# Autodesk Inventor assembly: MaleHeader-02
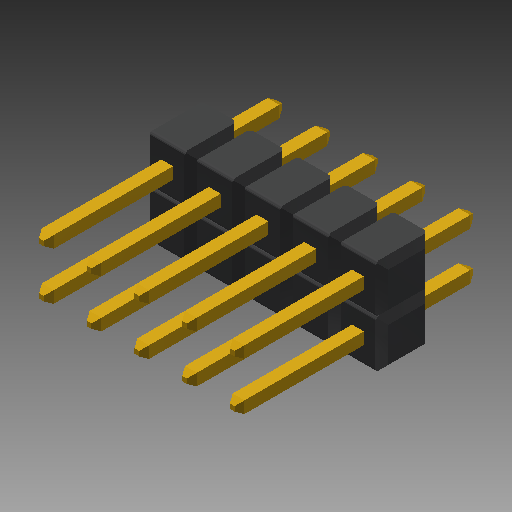
[picture p0: Inventor's stored thumbnail of the model, 512x512]
Saved by Autodesk Inventor 2018 (Build 220112000, 112)
## iProperties
Created: 2017-04-09
Part Number: MaleHeader-02
Document SubType Name: Assembly
Designer: dkt01
Author: dkt01
## Documents named in this file (2)
- C:\Users\dktur\Dropbox\StackLightMonitor\CAD\MaleHeader-02.iam
- C:\Users\dktur\Dropbox\StackLightMonitor\CAD\MaleHeader-02.ipt
## Components (10 placed, 1 different names)
1. MaleHeader-02:1
2. MaleHeader-02:2
3. MaleHeader-02:3
4. MaleHeader-02:4
5. MaleHeader-02:5
6. MaleHeader-02:6
7. MaleHeader-02:7
8. MaleHeader-02:8
9. MaleHeader-02:9
10. MaleHeader-02:10
## Component patterns: (10 elements, first: MaleHeader-02:1)
